# Autodesk Inventor assembly: am14u3LongWithArmAndGripperV02
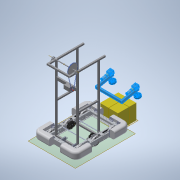
[picture p0: Inventor's stored thumbnail of the model, 180x180]
Saved by Autodesk Inventor 2022 (Build 260153000, 153)
## iProperties
Created: 2018-01-14
Part Number: am14u3LongWithArmAndGripperV02
Document SubType Name: Assembly
Designer: steele
Author: steele
## Documents named in this file (5)
- C:\git\CAD-Development\robSteele\2018-FRC\am14u3LongWithArmAndGripperV02.iam
- C:\git\CAD-Development\robSteele\2018-FRC\AMbaseLongWithBumper\Long with Bumper\DB_DriveBaseLong_AM14U3_Bumpers and Battery Tray.iam
- C:\git\CAD-Development\robSteele\2018-FRC\Field Elements\Cube-GE-18124.ipt
- C:\git\CAD-Development\robSteele\2018-FRC\Gripper\gripperAssembly.iam
- C:\git\CAD-Development\robSteele\2018-FRC\Arm\ArmAndMotorV02.iam
## Components (4 placed, 4 different names)
1. DB_DriveBaseLong_AM14U3_Bumpers and Battery Tray:1 [sub-assembly] — Flush:2, Mate:7, Mate:8, Mate:9, Mate:10
2. Cube-GE-18124:1
3. gripperAssembly:1 [sub-assembly] — Mate:7
4. ArmAndMotorV02:1 [sub-assembly] — Mate:8, Mate:9, Mate:10
## Relationships (5: Mate 4, Flush 1)
- Flush:2 (50.8 mm): DB_DriveBaseLong_AM14U3_Bumpers and Battery Tray:1
- Mate:7: DB_DriveBaseLong_AM14U3_Bumpers and Battery Tray:1 ↔ gripperAssembly:1
- Mate:8 (127 mm): DB_DriveBaseLong_AM14U3_Bumpers and Battery Tray:1 ↔ ArmAndMotorV02:1
- Mate:9: DB_DriveBaseLong_AM14U3_Bumpers and Battery Tray:1 ↔ ArmAndMotorV02:1
- Mate:10: DB_DriveBaseLong_AM14U3_Bumpers and Battery Tray:1 ↔ ArmAndMotorV02:1
